# Autodesk Inventor assembly: V-Slot Tnut Delrin Dual Wheel Assembly
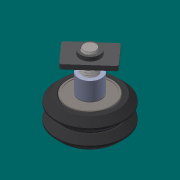
[picture p0: Inventor's stored thumbnail of the model, 180x180]
Saved by Autodesk Inventor 2016 (Build 200138000, 138)
## iProperties
Created: 2015-06-04
Part Number: V-Slot Tnut Delrin Dual Wheel Assembly
Document SubType Name: Assembly
Designer: Sawaiz Syed
Author: Sawaiz Syed
## Documents named in this file (7)
- C:\Users\Sawaiz\Documents\data\projects\cncBlackBox\vWheel\V-Slot Tnut Delrin Dual Wheel Assembly.iam
- C:\Users\Sawaiz\Documents\data\projects\cncBlackBox\hardware\delrinVWheel.ipt
- C:\Users\Sawaiz\Documents\data\projects\cncBlackBox\hardware\0.25inSpacer.ipt
- C:\Users\Sawaiz\Documents\data\projects\cncBlackBox\hardware\m5PrecisionWasher.ipt
- C:\Users\Sawaiz\Documents\data\projects\cncBlackBox\hardware\625BallBearing.ipt
- C:\Users\Sawaiz\Documents\data\projects\cncBlackBox\hardware\m5x25LowProfile.ipt
- C:\Users\Sawaiz\Documents\data\projects\cncBlackBox\hardware\m5TNut.ipt
## Components (7 placed, 6 different names)
1. delrinVWheel:1 — Mate:2, Flush:1, Mate:5, Mate:6
2. 0.25inSpacer:1 — Mate:1, Mate:3, Mate:4, Mate:7, Mate:8, Mate:11
3. m5PrecisionWasher:1 — Mate:3, Flush:1
4. 625BallBearing:1 — Mate:4, Mate:5, Mate:7
5. 625BallBearing:2 — Mate:1, Mate:2, Mate:6, Mate:9
6. m5x25LowProfile:1 — Mate:8, Mate:9, Mate:10
7. m5TNut:1 — Mate:10, Mate:11
## Relationships (12: Mate 11, Flush 1)
- Mate:1: 0.25inSpacer:1 ↔ 625BallBearing:2
- Mate:2: delrinVWheel:1 ↔ 625BallBearing:2
- Mate:3: 0.25inSpacer:1 ↔ m5PrecisionWasher:1
- Mate:4: 0.25inSpacer:1 ↔ 625BallBearing:1
- Flush:1: delrinVWheel:1 ↔ m5PrecisionWasher:1
- Mate:5: delrinVWheel:1 ↔ 625BallBearing:1
- Mate:6: delrinVWheel:1 ↔ 625BallBearing:2
- Mate:7: 0.25inSpacer:1 ↔ 625BallBearing:1
- Mate:8: 0.25inSpacer:1 ↔ m5x25LowProfile:1
- Mate:9: 625BallBearing:2 ↔ m5x25LowProfile:1
- Mate:10: m5x25LowProfile:1 ↔ m5TNut:1
- Mate:11 (4 mm): 0.25inSpacer:1 ↔ m5TNut:1
